# Autodesk Inventor assembly: ALL_03
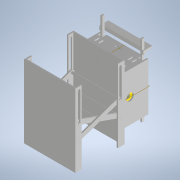
[picture p0: Inventor's stored thumbnail of the model, 180x180]
Saved by Autodesk Inventor 2020 (Build 240168000, 168)
## iProperties
Created: 2019-12-21
Part Number: ALL_03
Document SubType Name: Assembly
Designer: damien
Author: damien
## Documents named in this file (3)
- D:\fablab\save\Scisor\ALL_03.iam
- D:\fablab\save\Scisor\BOX_PART.iam
- D:\fablab\save\Scisor\table.iam
## Components (2 placed, 2 different names)
1. BOX_PART:1 [sub-assembly] — Affleurement:1, Affleurement:2, Affleurement:3, Affleurement:4, Placage:1, Placage:2
2. table:1 [sub-assembly] — Affleurement:4, Placage:1, Placage:2
## Relationships (6: Flush 4, Mate 2)
- Affleurement:1 [Flush]: BOX_PART:1
- Affleurement:2 [Flush]: BOX_PART:1
- Affleurement:3 [Flush]: BOX_PART:1
- Affleurement:4 [Flush]: BOX_PART:1 ↔ table:1
- Placage:1 [Mate]: BOX_PART:1 ↔ table:1
- Placage:2 [Mate]: BOX_PART:1 ↔ table:1
